# Autodesk Inventor assembly: Assembly_Casing
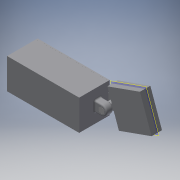
[picture p0: Inventor's stored thumbnail of the model, 180x180]
Saved by Autodesk Inventor 2019 (Build 230136000, 136)
## iProperties
Created: 2020-12-20
Part Number: Assembly_Casing
Document SubType Name: Assembly
Designer: nicolas
Author: nicolas
## Documents named in this file (7)
- C:\Workspace\3D\Cad\LampeSolaire2\Assembly_Casing.iam
- C:\Workspace\3D\Cad\LampeSolaire2\Casing_Part1.ipt
- C:\Workspace\3D\Cad\LampeSolaire2\Casing_Part2.ipt
- C:\Workspace\3D\Cad\LampeSolaire2\Casing_Part3.ipt
- C:\Workspace\3D\Cad\Screws\Hex_m5\M5x0.8xL\M5x0.8x25.ipt
- C:\Workspace\3D\Cad\Screws\Hex_m5\M5x0.8xL.ipt
- C:\Workspace\3D\Cad\Screws\wing_nuts\WNM5.ipt
## Components (5 placed, 5 different names)
1. Casing_Part1:1 — Flush:1, Cylindrical:1, Cylindrical:2, Mate:2, Mate:3
2. Casing_Part2:1 — Flush:1, Cylindrical:1, Mate:1, Mate:5
3. Casing_Part3:1 — Cylindrical:2
4. M5x0.8x25:1 — Mate:1, Mate:2, Mate:3, Mate:4
5. WNM5:1 — Mate:4, Mate:5
## Relationships (8: Mate 5, CylindricalJoint 2, Flush 1)
- Flush:1: Casing_Part1:1 ↔ Casing_Part2:1
- Cylindrical:1: Casing_Part1:1 ↔ Casing_Part2:1
- Cylindrical:2: Casing_Part1:1 ↔ Casing_Part3:1
- Mate:1: Casing_Part2:1 ↔ M5x0.8x25:1
- Mate:2: Casing_Part1:1 ↔ M5x0.8x25:1
- Mate:3: Casing_Part1:1 ↔ M5x0.8x25:1
- Mate:4: M5x0.8x25:1 ↔ WNM5:1
- Mate:5: Casing_Part2:1 ↔ WNM5:1
